# Autodesk Inventor assembly: cylinder_45001223510555_0
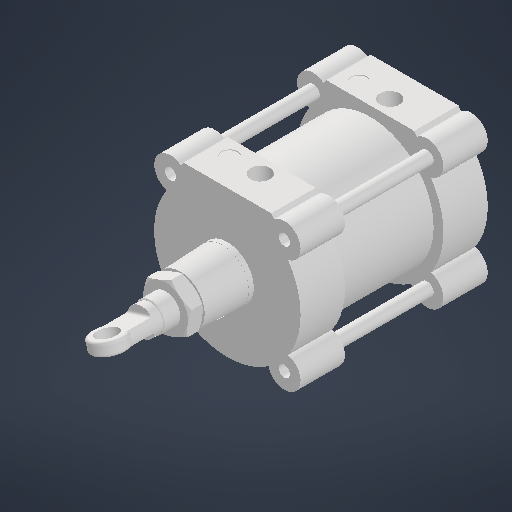
[picture p0: Inventor's stored thumbnail of the model, 512x512]
Saved by Autodesk Inventor 2025 (Build 290162000, 162)
## iProperties
Company: TraceParts S.A.
Created: 2024-05-27
Part Number: cylinder_45001223510555_0
Checked By: TraceParts S.A.
Catalog Web Link: www.traceparts.com
Document SubType Name: Assembly
Designer: TraceParts
Sending System: TraceParts v2
Major Version: 6.0
Minor Version: 0.0
Format Version: 0.0
Product Id: TraceParts v2
REFERENCE: 45001223510555
STANDARD: ISO 15552, AFNOR NF ISO 15552, DIN ISO 15552, ISO 6431, AFNOR NFE 49003, VDMA 24562
SUPPLIER: ASCO
DESIGN: PES cylinder with FPM rod seal, tie-rods, barrel aluminium, single rod, cushioned, equipped for detectors, bore 160 mm, stroke 50 mm
TraceParts.PartNumber: 10-31102002-070508
TraceParts.PartTitle: Double acting cylinder Ø 32 to 200 mm - 450 series - type PES (with tie rods) with rod seal only of FPM
TraceParts.InstanceId: 10-31102002-070508CBIB3JD51C785F3IUZ06YAQKU
TRACEPARTS: TRACEPARTS
TraceParts.PartLanguage: en
TraceParts.PartVersion: 1.7.5
Author: TraceParts
## Documents named in this file (5)
- D:\UNAL\2024-1S\APM\Digital Factory\Pneumatic Cylinders and Guides\cylinder_45001223510555_0.iam
- D:\UNAL\2024-1S\APM\Digital Factory\Pneumatic Cylinders and Guides\cylinder_45001223510555_0_01.ipt
- D:\UNAL\2024-1S\APM\Digital Factory\Pneumatic Cylinders and Guides\cylinder_45001223510555_0_02.ipt
- D:\UNAL\2024-1S\APM\Digital Factory\Pneumatic Cylinders and Guides\cylinder_45001223510555_0_03.ipt
- D:\UNAL\2024-1S\APM\Digital Factory\Packaging Machine\Ring.ipt
## Components (4 placed, 4 different names)
1. cylinder_45001223510555_0_Temp_1:1 — Cylindrical:1, Mate:1
2. cylinder_45001223510555_0_Temp_2:1 — Cylindrical:1, Rigid:1, Flush:1, Flush:2
3. cylinder_45001223510555_0_Temp_3:1 — Rigid:1, Mate:1
4. Ring:1 — Flush:1, Flush:2
## Relationships (5: Flush 2, CylindricalJoint 1, WeldJoint 1, Mate 1)
- Cylindrical:1: cylinder_45001223510555_0_Temp_1:1 ↔ cylinder_45001223510555_0_Temp_2:1
- Rigid:1 [WeldJoint]: cylinder_45001223510555_0_Temp_2:1 ↔ cylinder_45001223510555_0_Temp_3:1
- Flush:1: cylinder_45001223510555_0_Temp_2:1 ↔ Ring:1
- Flush:2: cylinder_45001223510555_0_Temp_2:1 ↔ Ring:1
- Mate:1: cylinder_45001223510555_0_Temp_1:1 ↔ cylinder_45001223510555_0_Temp_3:1
